# Autodesk Inventor assembly: Clevis-Socket
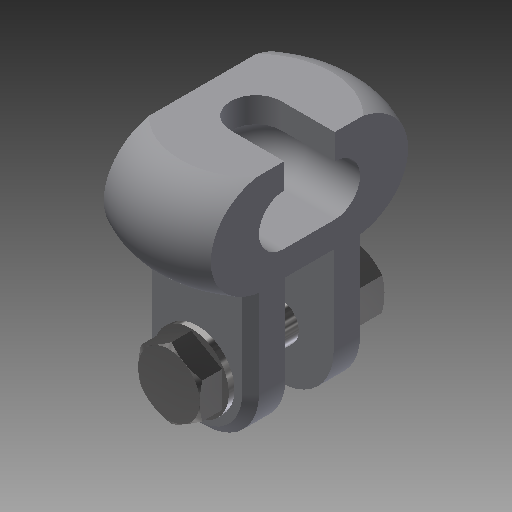
[picture p0: Inventor's stored thumbnail of the model, 512x512]
Saved by Autodesk Inventor 2018 (Build 220112000, 112)
## iProperties
Created: 2021-04-28
Part Number: Clevis-Socket
Document SubType Name: Assembly
Designer: l01767
Author: l01767
## Documents named in this file (3)
- C:\Users\l08619\Documents\Projetos\TAESA\Modelo 3D - Tensionadores e Suspensão\Suporte de Suspenção\Clevis-Socket.iam
- C:\Users\l08619\Documents\Projetos\TAESA\Modelo 3D - Tensionadores e Suspensão\Suporte de Suspenção\Clevis-Socket.ipt
- C:\Users\l08619\Documents\Projetos\TAESA\Modelo 3D - Tensionadores e Suspensão\Suporte de Suspenção\Bolted Connection1.iam
## Components (2 placed, 2 different names)
1. Clevis-Socket:1 — Mate:1, Mate:2
2. Bolted Connection:1 [sub-assembly] — Mate:1, Mate:2
## Relationships (2: Mate 2)
- Mate:1: Clevis-Socket:1 ↔ Bolted Connection:1
- Mate:2: Clevis-Socket:1 ↔ Bolted Connection:1
